# Autodesk Inventor assembly: Case_Assembly
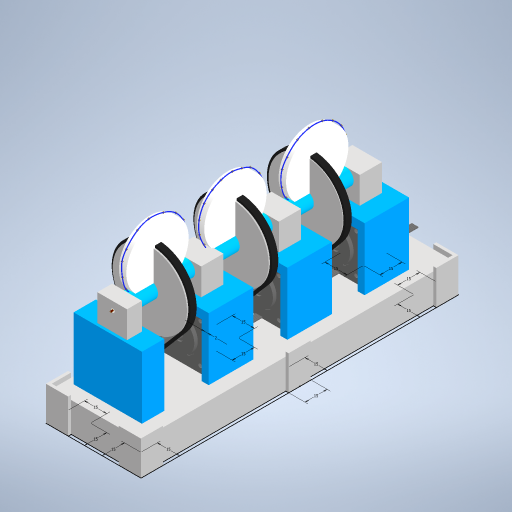
[picture p0: Inventor's stored thumbnail of the model, 512x512]
Saved by Autodesk Inventor 2024 (Build 280153000, 153)
## iProperties
Created: 2024-02-15
Part Number: Case_Assembly
Document SubType Name: Assembly
Designer: fabiancastano
Author: fabiancastano
## Documents named in this file (3)
- C:\GitHub\PulseLaserPrj\CaseDesign\Case_Assembly.iam
- C:\GitHub\PulseLaserPrj\CaseDesign\Polarizer.iam
- C:\GitHub\PulseLaserPrj\CaseDesign\Case_parts\BaseMotor.ipt
## Components (2 placed, 2 different names)
1. Polarizer:1 [sub-assembly] — Flush:1
2. BaseMotor:1 — Flush:1
## Relationships (1: Flush 1)
- Flush:1: Polarizer:1 ↔ BaseMotor:1
